# Autodesk Inventor assembly: __VK_WT_ZSB
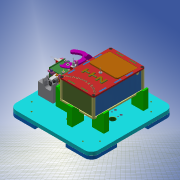
[picture p0: Inventor's stored thumbnail of the model, 180x180]
Saved by Autodesk Inventor 2019 (Build 230136000, 136)
## iProperties
Created: 2023-11-18
Part Number: __VK_WT_ZSB
Material: Generisch
Document SubType Name: Assembly
Designer: RP
Author: RP
## Documents named in this file (4)
- C:\Users\RP\Documents\Inventor\___Projekt_Useless_Box\_Verkettung\__VK_WT_beladen.iam
- C:\Users\RP\Documents\Inventor\___Projekt_Useless_Box\_Verkettung\__VK_WT.iam
- C:\Users\RP\Documents\Inventor\___Projekt_Useless_Box\_Useless_Box\Useless_Box.iam
- C:\Users\RP\Documents\Inventor\___Projekt_Useless_Box\_Useless_Box\Antriebseinheit_ZSB.iam
## Components (4 placed, 3 different names)
1. __VK_WT:1 [sub-assembly] — Fluchtend:16, Fluchtend:17, Fluchtend:18, Passend:12
2. Useless_Box:1 [sub-assembly] — Passend:12, Fluchtend:28
3. Antriebseinheit_ZSB:1 [sub-assembly] — Fluchtend:28
4. Antriebseinheit_ZSB:2 [sub-assembly]
## Relationships (20: Mate 15, Flush 5)
- [Flush]: __VK_WT:1
- [Mate]: __VK_WT:1
- [Mate] (20.3 mm): __VK_WT:1
- Fluchtend:16 [Flush]: __VK_WT:1
- Fluchtend:17 [Flush]: __VK_WT:1
- Fluchtend:18 [Flush]: __VK_WT:1
- [Mate]: __VK_WT:1 ↔ Useless_Box:1
- [Mate]: __VK_WT:1 ↔ Useless_Box:1
- Passend:12 [Mate]: __VK_WT:1 ↔ Useless_Box:1
- [Mate]: __VK_WT:1 ↔ Antriebseinheit_ZSB:1
- [Mate]: __VK_WT:1 ↔ Antriebseinheit_ZSB:1
- [Mate]: __VK_WT:1 ↔ Antriebseinheit_ZSB:1
- [Mate]: __VK_WT:1 ↔ Antriebseinheit_ZSB:2
- [Mate]: __VK_WT:1 ↔ Antriebseinheit_ZSB:2
- [Mate]: __VK_WT:1 ↔ Antriebseinheit_ZSB:2
- [Mate]: __VK_WT:1 ↔ Antriebseinheit_ZSB:1
- [Mate]: __VK_WT:1 ↔ Antriebseinheit_ZSB:1
- [Mate]: __VK_WT:1 ↔ Antriebseinheit_ZSB:1
- [Mate]: __VK_WT:1 ↔ Antriebseinheit_ZSB:1
- Fluchtend:28 [Flush]: Useless_Box:1 ↔ Antriebseinheit_ZSB:1
